# Autodesk Inventor assembly: MIR_HbFinger01ForChild
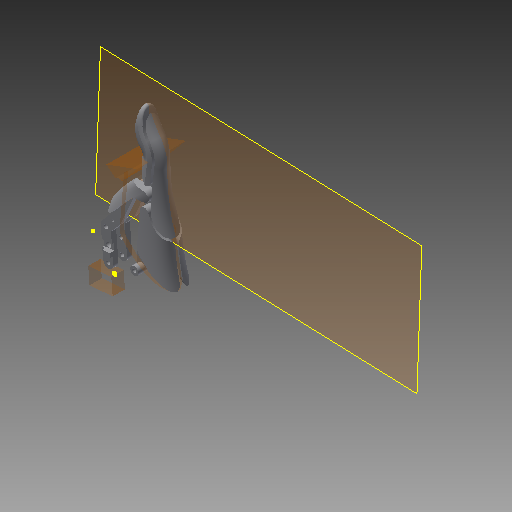
[picture p0: Inventor's stored thumbnail of the model, 512x512]
Saved by Autodesk Inventor 2018.1 (Build 221171000, 171)
## iProperties
Part Number: MIR_HbFinger01ForChild
Material: 一般
Document SubType Name: Assembly
Designer: sktom
Author: sktom
## Documents named in this file (8)
- D:\CloudStrage\OneDrive\CAD\MAJ\hackberry\HACKberry-hardware\3D_69%inlength\Inventor\HbHandForChild\HbFinger01ForChild\MIR_HbFinger01ForChild.iam
- D:\CloudStrage\OneDrive\CAD\MAJ\hackberry\HACKberry-hardware\3D_69%inlength\Inventor\HbHandForChild\HbFinger01ForChild\MIR_HbCouplerLinkCover03ForChild.ipt
- D:\CloudStrage\OneDrive\CAD\MAJ\hackberry\HACKberry-hardware\3D_69%inlength\Inventor\HbHandForChild\HbFinger01ForChild\MIR_HbCouplerLink02ForChild.ipt
- D:\CloudStrage\OneDrive\CAD\MAJ\hackberry\HACKberry-hardware\3D_69%inlength\Inventor\HbHandForChild\HbFinger01ForChild\MIR_HbMiddle-DistalPhalanx02ForChild.ipt
- D:\CloudStrage\OneDrive\CAD\MAJ\hackberry\HACKberry-hardware\3D_69%inlength\Inventor\HbHandForChild\HbFinger01ForChild\MIR_HbProximalPhalanx02ForChild.ipt
- D:\CloudStrage\OneDrive\CAD\MAJ\hackberry\HACKberry-hardware\3D_69%inlength\Inventor\HbHandForChild\HbFinger01ForChild\MIR_HbProximalPhalanxCover02ForChild.ipt
- D:\CloudStrage\OneDrive\CAD\MAJ\hackberry\HACKberry-hardware\3D_69%inlength\Inventor\HbHandForChild\HbFinger01ForChild\MIR_shaft_phi1.5_l6.ipt
- D:\CloudStrage\OneDrive\CAD\MAJ\hackberry\HACKberry-hardware\3D_69%inlength\Inventor\HbHandForChild\HbFinger01ForChild\MIR_bolt_M1.4L6.ipt
## Components (11 placed, 7 different names)
1. MIR_HbCouplerLinkCover03ForChild:1 — 挿入:9, 挿入:8, 挿入:7
2. MIR_HbCouplerLink02ForChild:1 — 挿入:9, 挿入:8, 挿入:11, 挿入:12
3. MIR_HbMiddle-DistalPhalanx02ForChild:1 — 挿入:7, 挿入:10, リジッド:2
4. MIR_HbProximalPhalanx02ForChild:1 — 挿入:6, 挿入:5
5. MIR_HbProximalPhalanxCover02ForChild:1 — 挿入:10, 挿入:6, 挿入:5, 挿入:13, 挿入:14
6. MIR_shaft_phi1.5_l6:1
7. MIR_shaft_phi1.5_l6:2 — リジッド:2
8. MIR_bolt_M1.4L6:1 — 挿入:11
9. MIR_bolt_M1.4L6:2 — 挿入:12
10. MIR_bolt_M1.4L6:3 — 挿入:13
11. MIR_bolt_M1.4L6:4 — 挿入:14
## Relationships (11: Insert 10, WeldJoint 1)
- 挿入:9 [Insert]: MIR_HbCouplerLinkCover03ForChild:1 ↔ MIR_HbCouplerLink02ForChild:1
- 挿入:8 [Insert]: MIR_HbCouplerLinkCover03ForChild:1 ↔ MIR_HbCouplerLink02ForChild:1
- 挿入:7 [Insert] (0.05 mm): MIR_HbCouplerLinkCover03ForChild:1 ↔ MIR_HbMiddle-DistalPhalanx02ForChild:1
- 挿入:10 [Insert] (0.1 mm): MIR_HbMiddle-DistalPhalanx02ForChild:1 ↔ MIR_HbProximalPhalanxCover02ForChild:1
- 挿入:6 [Insert]: MIR_HbProximalPhalanx02ForChild:1 ↔ MIR_HbProximalPhalanxCover02ForChild:1
- 挿入:5 [Insert]: MIR_HbProximalPhalanx02ForChild:1 ↔ MIR_HbProximalPhalanxCover02ForChild:1
- 挿入:11 [Insert]: MIR_HbCouplerLink02ForChild:1 ↔ MIR_bolt_M1.4L6:1
- 挿入:12 [Insert]: MIR_HbCouplerLink02ForChild:1 ↔ MIR_bolt_M1.4L6:2
- 挿入:13 [Insert]: MIR_HbProximalPhalanxCover02ForChild:1 ↔ MIR_bolt_M1.4L6:3
- 挿入:14 [Insert]: MIR_HbProximalPhalanxCover02ForChild:1 ↔ MIR_bolt_M1.4L6:4
- リジッド:2 [WeldJoint]: MIR_HbMiddle-DistalPhalanx02ForChild:1 ↔ MIR_shaft_phi1.5_l6:2
